# Autodesk Inventor assembly: Manipulator
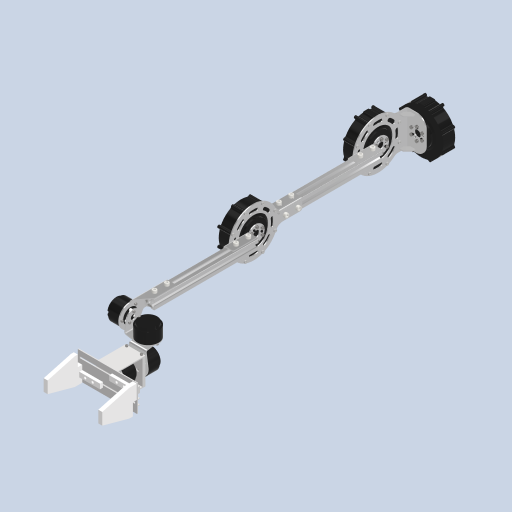
[picture p0: Inventor's stored thumbnail of the model, 512x512]
Saved by Autodesk Inventor 2023 (Build 270158000, 158)
## iProperties
Created: 2024-11-08
Part Number: Manipulator
Document SubType Name: Assembly
Designer: kiyo
Author: kiyo
## Documents named in this file (20)
- D:\GitHub\inventor\syu-si\OfficeRobot\Manipulator\Manipulator.iam
- D:\GitHub\inventor\syu-si\OfficeRobot\ReadyMade\Steadywin\GIM8108-8.iam
- D:\GitHub\inventor\syu-si\OfficeRobot\Manipulator\elbow-pitch-bracket.ipt
- D:\GitHub\inventor\syu-si\OfficeRobot\ReadyMade\Screw\M3_6mm.ipt
- D:\GitHub\inventor\syu-si\OfficeRobot\ReadyMade\Steadywin\GIM3505-8_with-driver.ipt
- D:\GitHub\inventor\syu-si\OfficeRobot\Manipulator\wrist_roll_plate.ipt
- D:\GitHub\inventor\syu-si\OfficeRobot\Manipulator\wrist-pitch-plate.ipt
- D:\GitHub\inventor\syu-si\OfficeRobot\ReadyMade\Screw\M2-5_6mm.ipt
- D:\GitHub\inventor\syu-si\OfficeRobot\ReadyMade\Screw\CBSH3-8.ipt
- D:\GitHub\inventor\syu-si\OfficeRobot\ReadyMade\Screw\FWSJJ-D5-V2_6-T4_5.ipt
- D:\GitHub\inventor\syu-si\OfficeRobot\ReadyMade\Screw\M2-5_10mm.ipt
- D:\GitHub\inventor\syu-si\OfficeRobot\ReadyMade\Screw\HNTU5-5.ipt
- D:\GitHub\inventor\syu-si\OfficeRobot\Manipulator\pitch_plate_20mm.ipt
- D:\GitHub\inventor\syu-si\OfficeRobot\ReadyMade\Aluminum-frame\HFS5-2020-210-AV10-BV35-CV175-DV200.ipt
- D:\GitHub\inventor\syu-si\OfficeRobot\Manipulator\sholder_roll_bracket.ipt
- D:\GitHub\inventor\syu-si\OfficeRobot\ReadyMade\Screw\SCB5-22.ipt
- D:\GitHub\inventor\syu-si\OfficeRobot\ReadyMade\Screw\SCB5-8.ipt
- D:\GitHub\inventor\syu-si\OfficeRobot\Manipulator\Hand_tyokudou.iam
- D:\GitHub\inventor\syu-si\OfficeRobot\ReadyMade\Screw\PACK-SWSJJ10-6-0_3.ipt
- D:\GitHub\inventor\syu-si\OfficeRobot\Manipulator\wrist-yaw-plate.ipt
## Components (118 placed, 19 different names)
1. pitch_plate_20mm:1 — メイト:3, フラッシュ:1, 挿入:355, 挿入:356, 挿入:357, 挿入:358, 挿入:359, 挿入:360, 角度:47
2. pitch_plate_20mm:2 — 挿入:345, フラッシュ:3, 角度:40
3. sholder_roll_bracket:1 — 挿入:350, 挿入:361, 挿入:362, 挿入:363, 挿入:364, 挿入:365, 挿入:366, 挿入:414, 挿入:415
4. elbow-pitch-bracket:1 — 挿入:448, 挿入:449, 正接:4, 正接:5, フラッシュ:10, メイト:35, メイト:36
5. wrist-yaw-plate:1 — 挿入:456, 挿入:457, 挿入:458, 挿入:459
6. wrist-pitch-plate:1 — メイト:29, メイト:30, 正接:1, 正接:2, 正接:3, 挿入:437, 挿入:438, 挿入:439, 挿入:450, 挿入:451
7. wrist_roll_plate:2 — 挿入:402, 挿入:403, 挿入:404, 挿入:405, 挿入:406, 挿入:407, 挿入:452
8. Hand_tyokudou:1 [sub-assembly] — 挿入:431, 挿入:434, 挿入:435, 挿入:462, 角度:59, 角度:60
9. HFS5-2020-210-AV10-BV35-CV175-DV200:1 — メイト:3, フラッシュ:1, フラッシュ:9, 角度:37, メイト:23, メイト:24, メイト:31, 角度:49, メイト:32, 角度:50, メイト:33, メイト:34, フラッシュ:10
10. HFS5-2020-210-AV10-BV35-CV175-DV200:2 — フラッシュ:3, 挿入:351, 挿入:352, 角度:27, 角度:28, 挿入:353, 挿入:354, 角度:29, 角度:30, メイト:15, メイト:16, 角度:33, フラッシュ:5, メイト:17, メイト:18, 角度:34, フラッシュ:6, メイト:25, メイト:26, メイト:27, メイト:28, メイト:29, メイト:30
11. M3_6mm:1 — 挿入:337
12. M3_6mm:2 — 挿入:336
13. M3_6mm:3 — 挿入:334
14. M3_6mm:4 — 挿入:338
15. M3_6mm:5 — 挿入:339
16. M3_6mm:6 — 挿入:335
17. M3_6mm:7 — 挿入:358
18. M3_6mm:8 — 挿入:357
19. M3_6mm:9 — 挿入:355
20. M3_6mm:10 — 挿入:356
21. M3_6mm:11 — 挿入:359
22. M3_6mm:12 — 挿入:360
23. M3_6mm:13 — 挿入:361
24. M3_6mm:14 — 挿入:363
25. M3_6mm:15 — 挿入:362
26. M3_6mm:16 — 挿入:364
27. M3_6mm:17 — 挿入:365
28. M3_6mm:18 — 挿入:366
29. CBSH3-8:1 — 挿入:307
30. CBSH3-8:2 — 挿入:308
31. CBSH3-8:3 — 挿入:302
32. CBSH3-8:4 — 挿入:304, 挿入:415
33. CBSH3-8:5 — 挿入:309
34. CBSH3-8:6 — 挿入:303
35. CBSH3-8:7 — 挿入:305
36. CBSH3-8:8 — 挿入:306
37. CBSH3-8:9 — 挿入:332
38. CBSH3-8:10 — 挿入:327, 挿入:449
39. CBSH3-8:11 — 挿入:330
40. CBSH3-8:12 — 挿入:328
41. CBSH3-8:13 — 挿入:329
42. CBSH3-8:14 — 挿入:331
43. CBSH3-8:15 — 挿入:326
44. CBSH3-8:16 — 挿入:333
45. M2-5_6mm:16 — 挿入:439
46. M2-5_6mm:17 — 挿入:438
47. M2-5_6mm:18 — 挿入:437
48. M2-5_6mm:13
49. M2-5_6mm:14
50. M2-5_6mm:15
51. M2-5_10mm:7 — 挿入:402
52. M2-5_10mm:8 — 挿入:403
53. M2-5_10mm:9 — 挿入:404
54. M2-5_10mm:10 — 挿入:430
55. M2-5_10mm:11
56. M2-5_10mm:12
57. M2-5_10mm:13 — 挿入:453, 挿入:456
58. M2-5_10mm:15 — 挿入:454, 挿入:457
59. M2-5_10mm:14 — 挿入:455, 挿入:458
60. PACK-SWSJJ10-6-0_3:16 — メイト:31, メイト:35
61. PACK-SWSJJ10-6-0_3:17 — メイト:32
62. FWSJJ-D5-V2_6-T4_5:16 — 挿入:454
63. FWSJJ-D5-V2_6-T4_5:17 — 挿入:453
64. FWSJJ-D5-V2_6-T4_5:18 — 挿入:455
65. PACK-SWSJJ10-6-0_3:1 — 挿入:429
66. PACK-SWSJJ10-6-0_3:2 — 挿入:428
67. PACK-SWSJJ10-6-0_3:3 — 挿入:418
68. PACK-SWSJJ10-6-0_3:4 — 挿入:419
69. PACK-SWSJJ10-6-0_3:5 — 挿入:421, メイト:36
70. PACK-SWSJJ10-6-0_3:7 — 挿入:423
71. PACK-SWSJJ10-6-0_3:8 — 挿入:424
72. PACK-SWSJJ10-6-0_3:9 — 挿入:422
73. PACK-SWSJJ10-6-0_3:11 — 挿入:420
74. PACK-SWSJJ10-6-0_3:12 — 挿入:427
75. PACK-SWSJJ10-6-0_3:13 — 挿入:417
76. PACK-SWSJJ10-6-0_3:14 — 挿入:416
77. FWSJJ-D5-V2_6-T4_5:10 — 挿入:407
78. FWSJJ-D5-V2_6-T4_5:11 — 挿入:405
79. FWSJJ-D5-V2_6-T4_5:12 — 挿入:406
80. FWSJJ-D5-V2_6-T4_5:13 — 挿入:430, 挿入:431
81. FWSJJ-D5-V2_6-T4_5:14 — 挿入:434
82. FWSJJ-D5-V2_6-T4_5:15 — 挿入:435
83. HNTU5-5:27 — 角度:49, メイト:33
84. SCB5-8:13 — 正接:4
85. HNTU5-5:28 — 角度:50, メイト:34
86. SCB5-8:14 — 正接:5
87. HNTU5-5:22 — 挿入:412, メイト:27, メイト:28
88. SCB5-8:8 — 挿入:412, 正接:2, 挿入:429
89. HNTU5-5:23 — 挿入:411, メイト:25, メイト:26
90. SCB5-8:9 — 挿入:411, 正接:3, 挿入:428
91. SCB5-22:1 — 挿入:368, 挿入:418
92. SCB5-22:2 — 挿入:367, 挿入:419
93. SCB5-22:3 — 挿入:370, 挿入:421
94. SCB5-22:4 — 挿入:369, 挿入:420
95. SCB5-22:5 — 挿入:372, 挿入:423
96. SCB5-22:6 — 挿入:371, 挿入:422
97. SCB5-22:7 — 挿入:376, 挿入:416
98. SCB5-22:8 — 挿入:375, 正接:1, 挿入:417
99. SCB5-8:3 — 挿入:427
100. SCB5-8:4
101. SCB5-8:7 — 挿入:424
102. HNTU5-5:6 — 挿入:372
103. HNTU5-5:7 — 挿入:371
104. HNTU5-5:9 — 挿入:369
105. HNTU5-5:10 — 挿入:370
106. HNTU5-5:11 — 挿入:351, 角度:28, 挿入:367
107. HNTU5-5:12 — 挿入:352, 角度:27, 挿入:368
108. HNTU5-5:13 — 挿入:353, 角度:30, 挿入:376
109. HNTU5-5:14 — 挿入:354, 角度:29, 挿入:375
110. HNTU5-5:17 — メイト:15, メイト:16, 角度:33, フラッシュ:5
111. HNTU5-5:18 — メイト:17, メイト:18, 角度:34, フラッシュ:6
112. HNTU5-5:21 — フラッシュ:9, 角度:37, メイト:23, メイト:24
113. GIM8108-8:1 [sub-assembly] — 挿入:350, 角度:54, 角度:55, 角度:58
114. GIM8108-8:2 [sub-assembly] — 挿入:302, 挿入:303, 挿入:304, 挿入:305, 挿入:306, 挿入:307, 挿入:308, 挿入:309, 挿入:414, 角度:47, 角度:55
115. GIM8108-8:3 [sub-assembly] — 挿入:326, 挿入:327, 挿入:328, 挿入:329, 挿入:330, 挿入:331, 挿入:332, 挿入:333, 挿入:334, 挿入:335, 挿入:336, 挿入:337, 挿入:338, 挿入:339, 挿入:345, 角度:40, 挿入:448
116. GIM3505-8_with-driver:9 — 挿入:450, 挿入:451, 挿入:452
117. GIM3505-8_with-driver:8 — 挿入:459
118. GIM3505-8_with-driver:10 — 挿入:462
## Relationships (165: Insert 111, Mate 22, Angle 21, Flush 6, Tangent 5)
- 挿入:302 [Insert] (2 mm): CBSH3-8:3 ↔ GIM8108-8:2
- 挿入:303 [Insert] (2 mm): CBSH3-8:6 ↔ GIM8108-8:2
- 挿入:304 [Insert] (2 mm): CBSH3-8:4 ↔ GIM8108-8:2
- 挿入:305 [Insert] (2 mm): CBSH3-8:7 ↔ GIM8108-8:2
- 挿入:306 [Insert] (2 mm): CBSH3-8:8 ↔ GIM8108-8:2
- 挿入:307 [Insert] (2 mm): CBSH3-8:1 ↔ GIM8108-8:2
- 挿入:308 [Insert] (2 mm): CBSH3-8:2 ↔ GIM8108-8:2
- 挿入:309 [Insert] (2 mm): CBSH3-8:5 ↔ GIM8108-8:2
- [Insert] (-0.75 mm): HFS5-2020-210-AV10-BV35-CV175-DV200:1 ↔ HNTU5-5:6
- [Angle] (0 deg): HFS5-2020-210-AV10-BV35-CV175-DV200:1 ↔ HNTU5-5:6
- [Insert] (-0.75 mm): HFS5-2020-210-AV10-BV35-CV175-DV200:1 ↔ HNTU5-5:7
- [Angle] (0 deg): HFS5-2020-210-AV10-BV35-CV175-DV200:1 ↔ HNTU5-5:7
- [Angle] (0 deg): HFS5-2020-210-AV10-BV35-CV175-DV200:1 ↔ HNTU5-5:6
- 挿入:326 [Insert] (2 mm): CBSH3-8:15 ↔ GIM8108-8:3
- 挿入:327 [Insert] (2 mm): CBSH3-8:10 ↔ GIM8108-8:3
- 挿入:328 [Insert] (2 mm): CBSH3-8:12 ↔ GIM8108-8:3
- 挿入:329 [Insert] (2 mm): CBSH3-8:13 ↔ GIM8108-8:3
- 挿入:330 [Insert] (2 mm): CBSH3-8:11 ↔ GIM8108-8:3
- 挿入:331 [Insert] (2 mm): CBSH3-8:14 ↔ GIM8108-8:3
- 挿入:332 [Insert] (2 mm): CBSH3-8:9 ↔ GIM8108-8:3
- 挿入:333 [Insert] (2 mm): CBSH3-8:16 ↔ GIM8108-8:3
- 挿入:334 [Insert] (2 mm): M3_6mm:3 ↔ GIM8108-8:3
- 挿入:335 [Insert] (2 mm): M3_6mm:6 ↔ GIM8108-8:3
- 挿入:336 [Insert] (2 mm): M3_6mm:2 ↔ GIM8108-8:3
- 挿入:337 [Insert] (2 mm): M3_6mm:1 ↔ GIM8108-8:3
- 挿入:338 [Insert] (2 mm): M3_6mm:4 ↔ GIM8108-8:3
- 挿入:339 [Insert] (2 mm): M3_6mm:5 ↔ GIM8108-8:3
- [Insert]: pitch_plate_20mm:1 ↔ GIM8108-8:2
- [Mate] (0.3 mm): pitch_plate_20mm:1 ↔ HFS5-2020-210-AV10-BV35-CV175-DV200:1
- メイト:3 [Mate] (0.3 mm): pitch_plate_20mm:1 ↔ HFS5-2020-210-AV10-BV35-CV175-DV200:1
- [Angle] (0 deg): HFS5-2020-210-AV10-BV35-CV175-DV200:1 ↔ HNTU5-5:9
- [Angle] (0 deg): HFS5-2020-210-AV10-BV35-CV175-DV200:1 ↔ HNTU5-5:10
- [Insert] (-0.75 mm): HFS5-2020-210-AV10-BV35-CV175-DV200:1 ↔ HNTU5-5:9
- [Insert] (-0.75 mm): HFS5-2020-210-AV10-BV35-CV175-DV200:1 ↔ HNTU5-5:10
- 挿入:345 [Insert]: pitch_plate_20mm:2 ↔ GIM8108-8:3
- [Mate] (0.3 mm): pitch_plate_20mm:2 ↔ HFS5-2020-210-AV10-BV35-CV175-DV200:2
- [Mate] (0.3 mm): pitch_plate_20mm:2 ↔ HFS5-2020-210-AV10-BV35-CV175-DV200:2
- 挿入:350 [Insert]: sholder_roll_bracket:1 ↔ GIM8108-8:1
- フラッシュ:1 [Flush]: pitch_plate_20mm:1 ↔ HFS5-2020-210-AV10-BV35-CV175-DV200:1
- フラッシュ:3 [Flush]: pitch_plate_20mm:2 ↔ HFS5-2020-210-AV10-BV35-CV175-DV200:2
- 挿入:351 [Insert] (-0.75 mm): HFS5-2020-210-AV10-BV35-CV175-DV200:2 ↔ HNTU5-5:11
- 挿入:352 [Insert] (-0.75 mm): HFS5-2020-210-AV10-BV35-CV175-DV200:2 ↔ HNTU5-5:12
- 角度:27 [Angle] (0 deg): HFS5-2020-210-AV10-BV35-CV175-DV200:2 ↔ HNTU5-5:12
- 角度:28 [Angle] (0 deg): HFS5-2020-210-AV10-BV35-CV175-DV200:2 ↔ HNTU5-5:11
- 挿入:353 [Insert] (-0.75 mm): HFS5-2020-210-AV10-BV35-CV175-DV200:2 ↔ HNTU5-5:13
- 挿入:354 [Insert] (-0.75 mm): HFS5-2020-210-AV10-BV35-CV175-DV200:2 ↔ HNTU5-5:14
- 角度:29 [Angle] (0 deg): HFS5-2020-210-AV10-BV35-CV175-DV200:2 ↔ HNTU5-5:14
- 角度:30 [Angle] (0 deg): HFS5-2020-210-AV10-BV35-CV175-DV200:2 ↔ HNTU5-5:13
- 挿入:355 [Insert]: pitch_plate_20mm:1 ↔ M3_6mm:9
- 挿入:356 [Insert]: pitch_plate_20mm:1 ↔ M3_6mm:10
- 挿入:357 [Insert]: pitch_plate_20mm:1 ↔ M3_6mm:8
- 挿入:358 [Insert]: pitch_plate_20mm:1 ↔ M3_6mm:7
- 挿入:359 [Insert]: pitch_plate_20mm:1 ↔ M3_6mm:11
- 挿入:360 [Insert]: pitch_plate_20mm:1 ↔ M3_6mm:12
- 挿入:361 [Insert]: sholder_roll_bracket:1 ↔ M3_6mm:13
- 挿入:362 [Insert]: sholder_roll_bracket:1 ↔ M3_6mm:15
- 挿入:363 [Insert]: sholder_roll_bracket:1 ↔ M3_6mm:14
- 挿入:364 [Insert]: sholder_roll_bracket:1 ↔ M3_6mm:16
- 挿入:365 [Insert]: sholder_roll_bracket:1 ↔ M3_6mm:17
- 挿入:366 [Insert]: sholder_roll_bracket:1 ↔ M3_6mm:18
- 挿入:367 [Insert] (-0.95 mm): SCB5-22:2 ↔ HNTU5-5:11
- 挿入:368 [Insert] (-0.95 mm): SCB5-22:1 ↔ HNTU5-5:12
- 挿入:369 [Insert] (-0.95 mm): SCB5-22:4 ↔ HNTU5-5:9
- 挿入:370 [Insert] (-0.95 mm): SCB5-22:3 ↔ HNTU5-5:10
- 挿入:371 [Insert] (-0.95 mm): SCB5-22:6 ↔ HNTU5-5:7
- 挿入:372 [Insert] (-0.95 mm): SCB5-22:5 ↔ HNTU5-5:6
- 挿入:375 [Insert] (-0.95 mm): SCB5-22:8 ↔ HNTU5-5:14
- 挿入:376 [Insert] (-0.95 mm): SCB5-22:7 ↔ HNTU5-5:13
- [Insert] (3.5 mm): SCB5-8:3 ↔ HNTU5-5:17
- メイト:15 [Mate]: HFS5-2020-210-AV10-BV35-CV175-DV200:2 ↔ HNTU5-5:17
- メイト:16 [Mate] (1 mm): HFS5-2020-210-AV10-BV35-CV175-DV200:2 ↔ HNTU5-5:17
- 角度:33 [Angle] (0 deg): HFS5-2020-210-AV10-BV35-CV175-DV200:2 ↔ HNTU5-5:17
- フラッシュ:5 [Flush] (33.5 mm): HFS5-2020-210-AV10-BV35-CV175-DV200:2 ↔ HNTU5-5:17
- [Insert] (3.2 mm): SCB5-8:4 ↔ HNTU5-5:18
- メイト:17 [Mate]: HFS5-2020-210-AV10-BV35-CV175-DV200:2 ↔ HNTU5-5:18
- メイト:18 [Mate] (1 mm): HFS5-2020-210-AV10-BV35-CV175-DV200:2 ↔ HNTU5-5:18
- 角度:34 [Angle] (0 deg): HFS5-2020-210-AV10-BV35-CV175-DV200:2 ↔ HNTU5-5:18
- フラッシュ:6 [Flush] (33.5 mm): HFS5-2020-210-AV10-BV35-CV175-DV200:2 ↔ HNTU5-5:18
- [Insert] (3.5 mm): SCB5-8:7 ↔ HNTU5-5:21
- フラッシュ:9 [Flush] (33.5 mm): HFS5-2020-210-AV10-BV35-CV175-DV200:1 ↔ HNTU5-5:21
- 角度:37 [Angle] (0 deg): HFS5-2020-210-AV10-BV35-CV175-DV200:1 ↔ HNTU5-5:21
- メイト:23 [Mate] (1 mm): HFS5-2020-210-AV10-BV35-CV175-DV200:1 ↔ HNTU5-5:21
- メイト:24 [Mate]: HFS5-2020-210-AV10-BV35-CV175-DV200:1 ↔ HNTU5-5:21
- 角度:40 [Angle] (0 deg): pitch_plate_20mm:2 ↔ GIM8108-8:3
- [Insert]: wrist_roll_plate:2 ↔ M2-5_6mm:13
- [Insert]: wrist_roll_plate:2 ↔ M2-5_6mm:14
- [Insert]: wrist_roll_plate:2 ↔ M2-5_6mm:15
- [Insert]: wrist_roll_plate:2 ↔ GIM3505-8_with-driver:8
- [Insert]: wrist_roll_plate:2 ↔ GIM3505-8_with-driver:8
- 挿入:402 [Insert]: wrist_roll_plate:2 ↔ M2-5_10mm:7
- 挿入:403 [Insert]: wrist_roll_plate:2 ↔ M2-5_10mm:8
- 挿入:404 [Insert]: wrist_roll_plate:2 ↔ M2-5_10mm:9
- 挿入:405 [Insert]: wrist_roll_plate:2 ↔ FWSJJ-D5-V2_6-T4_5:11
- 挿入:406 [Insert]: wrist_roll_plate:2 ↔ FWSJJ-D5-V2_6-T4_5:12
- 挿入:407 [Insert]: wrist_roll_plate:2 ↔ FWSJJ-D5-V2_6-T4_5:10
- 挿入:411 [Insert] (3.5 mm): HNTU5-5:23 ↔ SCB5-8:9
- 挿入:412 [Insert] (3.5 mm): HNTU5-5:22 ↔ SCB5-8:8
- メイト:25 [Mate]: HFS5-2020-210-AV10-BV35-CV175-DV200:2 ↔ HNTU5-5:23
- メイト:26 [Mate] (1 mm): HFS5-2020-210-AV10-BV35-CV175-DV200:2 ↔ HNTU5-5:23
- メイト:27 [Mate] (1 mm): HFS5-2020-210-AV10-BV35-CV175-DV200:2 ↔ HNTU5-5:22
- メイト:28 [Mate]: HFS5-2020-210-AV10-BV35-CV175-DV200:2 ↔ HNTU5-5:22
- メイト:29 [Mate] (0.3 mm): wrist-pitch-plate:1 ↔ HFS5-2020-210-AV10-BV35-CV175-DV200:2
- メイト:30 [Mate] (0.3 mm): wrist-pitch-plate:1 ↔ HFS5-2020-210-AV10-BV35-CV175-DV200:2
- 正接:1 [Tangent] (0.25 mm): wrist-pitch-plate:1 ↔ SCB5-22:8
- 正接:2 [Tangent] (0.25 mm): wrist-pitch-plate:1 ↔ SCB5-8:8
- 正接:3 [Tangent] (0.25 mm): wrist-pitch-plate:1 ↔ SCB5-8:9
- 挿入:414 [Insert]: sholder_roll_bracket:1 ↔ GIM8108-8:2
- 挿入:415 [Insert]: sholder_roll_bracket:1 ↔ CBSH3-8:4
- 角度:47 [Angle] (0 deg): pitch_plate_20mm:1 ↔ GIM8108-8:2
- 挿入:416 [Insert] (2 mm): PACK-SWSJJ10-6-0_3:14 ↔ SCB5-22:7
- 挿入:417 [Insert] (2 mm): PACK-SWSJJ10-6-0_3:13 ↔ SCB5-22:8
- 挿入:418 [Insert] (2 mm): PACK-SWSJJ10-6-0_3:3 ↔ SCB5-22:1
- 挿入:419 [Insert] (2 mm): PACK-SWSJJ10-6-0_3:4 ↔ SCB5-22:2
- 挿入:420 [Insert] (2 mm): PACK-SWSJJ10-6-0_3:11 ↔ SCB5-22:4
- 挿入:421 [Insert] (2 mm): PACK-SWSJJ10-6-0_3:5 ↔ SCB5-22:3
- 挿入:422 [Insert] (2 mm): PACK-SWSJJ10-6-0_3:9 ↔ SCB5-22:6
- 挿入:423 [Insert] (2 mm): PACK-SWSJJ10-6-0_3:7 ↔ SCB5-22:5
- 挿入:424 [Insert] (2 mm): PACK-SWSJJ10-6-0_3:8 ↔ SCB5-8:7
- 挿入:427 [Insert] (2 mm): PACK-SWSJJ10-6-0_3:12 ↔ SCB5-8:3
- 挿入:428 [Insert] (2 mm): PACK-SWSJJ10-6-0_3:2 ↔ SCB5-8:9
- 挿入:429 [Insert] (2 mm): PACK-SWSJJ10-6-0_3:1 ↔ SCB5-8:8
- 挿入:430 [Insert] (2 mm): M2-5_10mm:10 ↔ FWSJJ-D5-V2_6-T4_5:13
- 挿入:431 [Insert]: Hand_tyokudou:1 ↔ FWSJJ-D5-V2_6-T4_5:13
- [Insert] (2 mm): M2-5_10mm:11 ↔ FWSJJ-D5-V2_6-T4_5:14
- [Insert] (2 mm): M2-5_10mm:12 ↔ FWSJJ-D5-V2_6-T4_5:15
- 挿入:434 [Insert]: Hand_tyokudou:1 ↔ FWSJJ-D5-V2_6-T4_5:14
- 挿入:435 [Insert]: Hand_tyokudou:1 ↔ FWSJJ-D5-V2_6-T4_5:15
- 挿入:437 [Insert]: wrist-pitch-plate:1 ↔ M2-5_6mm:18
- 挿入:438 [Insert]: wrist-pitch-plate:1 ↔ M2-5_6mm:17
- 挿入:439 [Insert]: wrist-pitch-plate:1 ↔ M2-5_6mm:16
- [Insert] (3.5 mm): HNTU5-5:27 ↔ SCB5-8:13
- [Insert] (3.5 mm): HNTU5-5:28 ↔ SCB5-8:14
- [Insert] (2 mm): PACK-SWSJJ10-6-0_3:17 ↔ SCB5-8:14
- [Insert] (2 mm): PACK-SWSJJ10-6-0_3:16 ↔ SCB5-8:13
- メイト:31 [Mate]: HFS5-2020-210-AV10-BV35-CV175-DV200:1 ↔ PACK-SWSJJ10-6-0_3:16
- 角度:49 [Angle] (0 deg): HFS5-2020-210-AV10-BV35-CV175-DV200:1 ↔ HNTU5-5:27
- メイト:32 [Mate]: HFS5-2020-210-AV10-BV35-CV175-DV200:1 ↔ PACK-SWSJJ10-6-0_3:17
- 角度:50 [Angle] (0 deg): HFS5-2020-210-AV10-BV35-CV175-DV200:1 ↔ HNTU5-5:28
- メイト:33 [Mate] (1 mm): HFS5-2020-210-AV10-BV35-CV175-DV200:1 ↔ HNTU5-5:27
- メイト:34 [Mate] (1 mm): HFS5-2020-210-AV10-BV35-CV175-DV200:1 ↔ HNTU5-5:28
- 挿入:448 [Insert]: elbow-pitch-bracket:1 ↔ GIM8108-8:3
- 挿入:449 [Insert]: elbow-pitch-bracket:1 ↔ CBSH3-8:10
- 正接:4 [Tangent] (0.25 mm): elbow-pitch-bracket:1 ↔ SCB5-8:13
- 正接:5 [Tangent] (0.25 mm): elbow-pitch-bracket:1 ↔ SCB5-8:14
- フラッシュ:10 [Flush]: elbow-pitch-bracket:1 ↔ HFS5-2020-210-AV10-BV35-CV175-DV200:1
- メイト:35 [Mate]: elbow-pitch-bracket:1 ↔ PACK-SWSJJ10-6-0_3:16
- メイト:36 [Mate]: elbow-pitch-bracket:1 ↔ PACK-SWSJJ10-6-0_3:5
- 挿入:450 [Insert]: wrist-pitch-plate:1 ↔ GIM3505-8_with-driver:9
- 挿入:451 [Insert]: wrist-pitch-plate:1 ↔ GIM3505-8_with-driver:9
- 挿入:452 [Insert] (4.5 mm): wrist_roll_plate:2 ↔ GIM3505-8_with-driver:9
- 挿入:453 [Insert] (2 mm): M2-5_10mm:13 ↔ FWSJJ-D5-V2_6-T4_5:17
- 挿入:454 [Insert] (2 mm): M2-5_10mm:15 ↔ FWSJJ-D5-V2_6-T4_5:16
- 挿入:455 [Insert] (2 mm): M2-5_10mm:14 ↔ FWSJJ-D5-V2_6-T4_5:18
- 挿入:456 [Insert]: wrist-yaw-plate:1 ↔ M2-5_10mm:13
- 挿入:457 [Insert]: wrist-yaw-plate:1 ↔ M2-5_10mm:15
- 挿入:458 [Insert]: wrist-yaw-plate:1 ↔ M2-5_10mm:14
- 挿入:459 [Insert] (4.5 mm): wrist-yaw-plate:1 ↔ GIM3505-8_with-driver:8
- [Insert]: wrist-yaw-plate:1 ↔ GIM3505-8_with-driver:10
- [Insert]: wrist-yaw-plate:1 ↔ GIM3505-8_with-driver:10
- 挿入:462 [Insert] (4.5 mm): Hand_tyokudou:1 ↔ GIM3505-8_with-driver:10
- 角度:54 [Angle] (0 deg): GIM8108-8:1
- 角度:55 [Angle] (180 deg): GIM8108-8:1 ↔ GIM8108-8:2
- 角度:58 [Angle] (180 deg): GIM8108-8:1
- 角度:59 [Angle] (0 deg): Hand_tyokudou:1
- 角度:60 [Angle] (0 deg): Hand_tyokudou:1
## Named parameters: d472_d466 = 3.5 mm, d477_d466 = 3.2 mm, d492_d466 = 3.5 mm, d516_d512 = 0 mm, d517_d513 = 0 mm, d519_d268 = 0 mm, d520_d269 = 0 mm, d521_d270 = 0 mm, d583_d581 = 2 mm, d584_d581 = 2 mm, d595_d482_d466 = 3.5 mm, d596_d483_d466 = 3.5 mm, d597_d576 = 2 mm, d598_d577 = 2 mm
